# Autodesk Inventor assembly: SERVO+GEARBOX ASSEMBLY_MIR
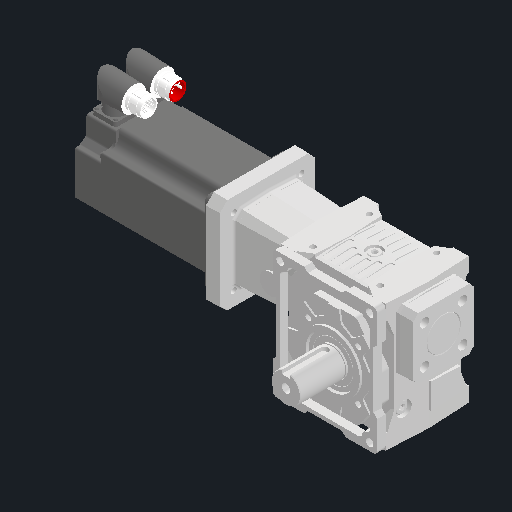
[picture p0: Inventor's stored thumbnail of the model, 512x512]
Saved by Autodesk Inventor 2025 (Build 290162000, 162)
## iProperties
Created: 2024-05-18
Part Number: SERVO+GEARBOX ASSEMBLY_MIR
Document SubType Name: Assembly
Designer: zulet
Author: zulet
## Documents named in this file (4)
- D:\UNAL\2024-1S\APM\Digital Factory\Packaging Machine\SERVO+GEARBOX ASSEMBLY_MIR.iam
- D:\UNAL\2024-1S\APM\Digital Factory\Worm Gear Boxes\148481481-9-dynabox_45_medium_p_h1_bm_f115-95_\dynabox_45_medium_p_h1_bm_f115-95__MIR.iam
- D:\UNAL\2024-1S\APM\Digital Factory\Motors\148481278-9-servo_motor_mpl_b430p_mk72aa\servo_motor_mpl_b430p_mk72aa_MIR.iam
- D:\UNAL\2024-1S\APM\Digital Factory\Packaging Machine\Servo-Gear-MountingPlate_MIR.ipt
## Components (3 placed, 3 different names)
1. dynabox_45_medium_p_h1_bm_f115-95__MIR:1 [sub-assembly] — Mate:2, Mate:1, Flush:1
2. servo_motor_mpl_b430p_mk72aa_MIR:1 [sub-assembly] — Mate:2, Mate:1
3. Servo-Gear-MountingPlate_MIR:1 — Flush:1
## Relationships (3: Mate 3)
- Mate:2: dynabox_45_medium_p_h1_bm_f115-95__MIR:1 ↔ servo_motor_mpl_b430p_mk72aa_MIR:1
- Mate:1: dynabox_45_medium_p_h1_bm_f115-95__MIR:1 ↔ servo_motor_mpl_b430p_mk72aa_MIR:1
- Flush:1 [Mate]: dynabox_45_medium_p_h1_bm_f115-95__MIR:1 ↔ Servo-Gear-MountingPlate_MIR:1
